# Autodesk Inventor assembly: Ensamble eléctrico
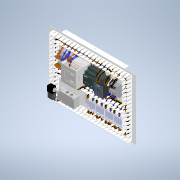
[picture p0: Inventor's stored thumbnail of the model, 180x180]
Saved by Autodesk Inventor 2021 (Build 250183000, 183)
## iProperties
Created: 2021-04-14
Part Number: Ensamble eléctrico
Document SubType Name: Assembly
Designer: Nelson
Mass: 3673.58 g
Surface Area: 11945 cm^2
Volume: 1889.25 cm^3
Density: 1.94447 g/cm^3
Author: Nelson
## Documents named in this file (23)
- C:\Users\Nelson\Github\Proyecto_PAI_2021\01 CAD\Ensamble eléctrico.iam
- C:\Users\Nelson\Github\Proyecto_PAI_2021\01 CAD\PLC-CP1E_N20DT1_D.iam
- C:\Users\Nelson\Github\Proyecto_PAI_2021\01 CAD\FuenteDC.iam
- C:\Users\Nelson\Github\Proyecto_PAI_2021\01 CAD\Rele de estado solido.ipt
- C:\Users\Nelson\Github\Proyecto_PAI_2021\01 CAD\Portafusible para fusible de 2A.ipt
- C:\Users\Nelson\Github\Proyecto_PAI_2021\01 CAD\Contactor.ipt
- C:\Users\Nelson\Github\Proyecto_PAI_2021\01 CAD\Riel 35x7.5 378mm.ipt
- C:\Users\Nelson\Github\Proyecto_PAI_2021\01 CAD\Bornera_AC.ipt
- C:\Users\Nelson\Github\Proyecto_PAI_2021\01 CAD\Bornera_DC.ipt
- C:\Users\Nelson\Github\Proyecto_PAI_2021\01 CAD\Canaleta 30x30 438mm.iam
- C:\Users\Nelson\Github\Proyecto_PAI_2021\01 CAD\Canaleta 30x30 378mm.iam
- C:\Users\Nelson\Github\Proyecto_PAI_2021\01 CAD\Canaleta 30x30 317mm.iam
- C:\Users\Nelson\Github\Proyecto_PAI_2021\01 CAD\Tapa_interior_1b.ipt
- C:\Users\Nelson\Github\Proyecto_PAI_2021\01 CAD\DIN EN ISO 7049 - ST4,8 x 13 - C - H.ipt
- C:\Users\Nelson\Github\Proyecto_PAI_2021\01 CAD\Ensamble electroválvula y bobina.iam
- C:\Users\Nelson\Github\Proyecto_PAI_2021\01 CAD\Fusible de 2A.ipt
- C:\Users\Nelson\Github\Proyecto_PAI_2021\01 CAD\Base Valvula.ipt
- C:\Users\Nelson\Github\Proyecto_PAI_2021\01 CAD\DIN EN ISO 7049 - ST4,8 x 38 - C - H.ipt
- C:\Users\Nelson\Github\Proyecto_PAI_2021\01 CAD\v70ss004001.iam
- C:\Users\Nelson\Github\Proyecto_PAI_2021\01 CAD\SV1.25-4S.ipt
- C:\Users\Nelson\Github\Proyecto_PAI_2021\01 CAD\v70ss004002.iam
- C:\Users\Nelson\Github\Proyecto_PAI_2021\01 CAD\Ensamble eléctrico\AIP\Cable and Harness\Ensamble eléctrico.Harness1.iam
- C:\Users\Nelson\Github\Proyecto_PAI_2021\01 CAD\1-34243-1.ipt
## Components (137 placed, 22 different names)
1. PLC-CP1E_N20DT1_D:1 [sub-assembly] — Mate:13, Mate:14, Mate:147, Mate:148, Mate:249, Mate:250, Mate:251, Mate:252, Mate:253, Mate:254, Mate:255, Mate:256, Mate:260, Mate:261, Mate:262, Mate:263, Mate:378, Mate:379, Mate:380, Mate:381, Mate:382, Mate:383, Mate:384, Mate:385, Mate:386, Mate:387, Mate:388, Mate:389, Mate:390, Mate:391, Mate:392, Mate:393, Mate:394, Mate:395, Mate:396, Mate:397, Mate:398, Mate:399, Mate:401, Mate:402, Mate:403, Mate:404, Mate:405, Mate:406, Mate:407, Mate:408, Mate:409, Mate:410, Mate:411
2. FuenteDC:1 [sub-assembly] — Mate:15, Mate:16, Mate:148, Mate:149, Mate:243, Mate:244, Mate:245, Mate:246, Mate:247, Mate:248, Mate:364, Mate:365, Mate:366, Mate:367, Mate:368, Mate:369
3. Portafusible para fusible de 2A:1 — Mate:17, Mate:18, Mate:149, Mate:150, Mate:204, Mate:205, Mate:360, Mate:361, Mate:362, Mate:363
4. Contactor:1 — Mate:19, Mate:20, Mate:150, Mate:151, Mate:370, Mate:371, Mate:372, Mate:373, Mate:374, Mate:375, Mate:376, Mate:377
5. Riel 35x7.5 378mm:1 — Mate:13, Mate:14, Mate:15, Mate:16, Mate:17, Mate:18, Mate:19, Mate:20, Mate:21, Mate:22, Mate:23, Mate:24, Mate:26, Mate:27, Mate:28, Mate:29, Mate:31, Mate:32, Mate:34, Mate:35, Mate:37, Mate:38, Mate:39, Mate:40, Mate:42, Mate:43, Mate:45, Mate:46, Mate:48, Mate:49, Mate:87, Mate:96, Mate:97, Flush:45, Mate:141, Mate:143, Mate:145, Mate:294, Mate:295, Mate:296, Mate:297, Mate:298, Mate:299, Mate:300, Mate:301
6. Bornera_AC:1 — Mate:21, Mate:22, Mate:25, Mate:151, Mate:338, Mate:339, Mate:343, Mate:359
7. Bornera_AC:2 — Mate:23, Mate:24, Mate:25, Mate:305, Mate:340, Mate:341, Mate:344, Mate:358
8. Bornera_DC:1 — Mate:26, Mate:27, Mate:30, Mate:89, Mate:215, Mate:222
9. Bornera_DC:2 — Mate:28, Mate:29, Mate:30, Mate:33, Mate:211, Mate:214, Mate:218, Mate:221
10. Bornera_DC:3 — Mate:31, Mate:32, Mate:33, Mate:36, Mate:210, Mate:213, Mate:217, Mate:220
11. Bornera_DC:4 — Mate:34, Mate:35, Mate:36, Mate:146, Mate:209, Mate:212, Mate:216, Mate:219
12. Bornera_DC:5 — Mate:39, Mate:40, Mate:41, Mate:44, Mate:226, Mate:231, Mate:236, Mate:241
13. Bornera_DC:6 — Mate:42, Mate:43, Mate:44, Mate:47, Mate:225, Mate:230, Mate:235, Mate:240
14. Bornera_DC:7 — Mate:45, Mate:46, Mate:47, Mate:50, Mate:224, Mate:229, Mate:234, Mate:239
15. Bornera_DC:8 — Mate:48, Mate:49, Mate:50, Mate:89, Mate:223, Mate:228, Mate:233, Mate:238
16. Bornera_DC:9 — Mate:37, Mate:38, Mate:41, Mate:147, Mate:227, Mate:232, Mate:237, Mate:242
17. Canaleta 30x30 438mm:1 [sub-assembly] — Mate:79, Mate:83, Mate:96, Flush:41, Mate:109, Flush:53, Mate:116, Mate:117, Mate:118, Mate:119, Mate:120, Mate:121
18. Canaleta 30x30 317mm:1 [sub-assembly] — Mate:79, Mate:81, Mate:87, Mate:94, Flush:41, Flush:42, Flush:54, Mate:110, Mate:111, Mate:112, Mate:113, Mate:114, Mate:115, Mate:146
19. Canaleta 30x30 438mm:2 [sub-assembly] — Mate:81, Mate:84, Flush:42, Flush:43, Mate:128, Mate:129, Mate:130, Mate:131, Mate:132, Mate:133, Mate:412, Flush:57, Mate:413, Flush:58, Mate:414, Mate:415
20. Canaleta 30x30 317mm:2 [sub-assembly] — Mate:83, Mate:84, Flush:43, Flush:44, Flush:45, Mate:122, Mate:123, Mate:124, Mate:125, Mate:126, Mate:127
21. Canaleta 30x30 378mm:1 [sub-assembly] — Mate:94, Mate:97, Flush:44, Mate:134, Mate:135, Mate:136, Mate:137, Mate:138, Mate:139
22. Tapa_interior_1b:1 — Flush:51, Flush:52, Mate:109, Flush:53, Flush:54, Mate:140, Mate:177, Mate:178, Mate:179, Mate:180, Mate:181, Mate:182, Mate:183, Mate:184, Mate:185, Mate:186, Mate:187, Mate:188, Coincidencia:206
23. DIN EN ISO 7049 - C-H ST4,8 x 13 - C - H:1 — Mate:110, Mate:111
24. DIN EN ISO 7049 - C-H ST4,8 x 13 - C - H:2 — Mate:112, Mate:113
25. DIN EN ISO 7049 - C-H ST4,8 x 13 - C - H:3 — Mate:114, Mate:115
26. DIN EN ISO 7049 - C-H ST4,8 x 13 - C - H:4 — Mate:122, Mate:123
27. DIN EN ISO 7049 - C-H ST4,8 x 13 - C - H:5 — Mate:124, Mate:125
28. DIN EN ISO 7049 - C-H ST4,8 x 13 - C - H:6 — Mate:126, Mate:127
29. DIN EN ISO 7049 - C-H ST4,8 x 13 - C - H:7 — Mate:132, Mate:133
30. DIN EN ISO 7049 - C-H ST4,8 x 13 - C - H:8 — Mate:130, Mate:131
31. DIN EN ISO 7049 - C-H ST4,8 x 13 - C - H:9 — Mate:128, Mate:129
32. DIN EN ISO 7049 - C-H ST4,8 x 13 - C - H:10 — Mate:116, Mate:117
33. DIN EN ISO 7049 - C-H ST4,8 x 13 - C - H:11 — Mate:118, Mate:119
34. DIN EN ISO 7049 - C-H ST4,8 x 13 - C - H:12 — Mate:120, Mate:121
35. DIN EN ISO 7049 - C-H ST4,8 x 13 - C - H:13 — Mate:138, Mate:139
36. DIN EN ISO 7049 - C-H ST4,8 x 13 - C - H:14 — Mate:136, Mate:137
37. DIN EN ISO 7049 - C-H ST4,8 x 13 - C - H:15 — Mate:134, Mate:135
38. DIN EN ISO 7049 - C-H ST4,8 x 13 - C - H:16 — Mate:140, Mate:141
39. DIN EN ISO 7049 - C-H ST4,8 x 13 - C - H:17 — Mate:143
40. DIN EN ISO 7049 - C-H ST4,8 x 13 - C - H:18 — Mate:145
41. Rele de estado solido:1 — Mate:177, Mate:178, Mate:179, Mate:189, Mate:190, Mate:191, Mate:192, Mate:306, Mate:307, Mate:314, Mate:315, Mate:322, Mate:323, Mate:336, Mate:337
42. Rele de estado solido:2 — Mate:180, Mate:181, Mate:182, Mate:193, Mate:194, Mate:195, Mate:308, Mate:309, Mate:316, Mate:317, Mate:324, Mate:325, Mate:334, Mate:335
43. Rele de estado solido:3 — Mate:183, Mate:184, Mate:185, Mate:196, Mate:197, Mate:198, Mate:199, Mate:310, Mate:311, Mate:318, Mate:319, Mate:326, Mate:327, Mate:332, Mate:333
44. Rele de estado solido:4 — Mate:186, Mate:187, Mate:188, Mate:200, Mate:201, Mate:202, Mate:203, Mate:312, Mate:313, Mate:320, Mate:321, Mate:328, Mate:329, Mate:330, Mate:331
45. DIN EN ISO 7049 - C-H ST4,8 x 13 - C - H:19 — Mate:189, Mate:190
46. DIN EN ISO 7049 - C-H ST4,8 x 13 - C - H:20 — Mate:191, Mate:192
47. DIN EN ISO 7049 - C-H ST4,8 x 13 - C - H:21 — Mate:193, Mate:194
48. DIN EN ISO 7049 - C-H ST4,8 x 13 - C - H:22 — Mate:195
49. DIN EN ISO 7049 - C-H ST4,8 x 13 - C - H:23 — Mate:196, Mate:197
50. DIN EN ISO 7049 - C-H ST4,8 x 13 - C - H:24 — Mate:198, Mate:199
51. DIN EN ISO 7049 - C-H ST4,8 x 13 - C - H:25 — Mate:200, Mate:201
52. DIN EN ISO 7049 - C-H ST4,8 x 13 - C - H:26 — Mate:202, Mate:203
53. Fusible de 2A:1 — Mate:204, Mate:205
54. Ensamble electroválvula y bobina:2 [sub-assembly] — Coincidencia:207, Nivelación:56, Coincidencia:208, De rotación:5, De rotación:6
55. Base Valvula:1 — Coincidencia:206, Coincidencia:207, Nivelación:56, Coincidencia:208, De rotación:1, De rotación:2, De rotación:3, De rotación:4
56. DIN EN ISO 7049 - C-H ST4,8 x 13 - C - H:27 — De rotación:1
57. DIN EN ISO 7049 - C-H ST4,8 x 13 - C - H:28 — De rotación:2
58. DIN EN ISO 7049 - C-H ST4,8 x 13 - C - H:29 — De rotación:4
59. DIN EN ISO 7049 - C-H ST4,8 x 13 - C - H:30 — De rotación:3
60. DIN EN ISO 7049 - C-H ST4,8 x 38 - C - H:1 — De rotación:6
61. DIN EN ISO 7049 - C-H ST4,8 x 38 - C - H:2 — De rotación:5
62. v70ss004001:1 [sub-assembly] — Mate:209, Mate:216
63. v70ss004001:2 [sub-assembly] — Mate:210, Mate:217
64. v70ss004001:3 [sub-assembly] — Mate:211, Mate:218
65. v70ss004001:4 [sub-assembly] — Mate:215, Mate:222
66. v70ss004001:5 [sub-assembly] — Mate:213, Mate:220
67. v70ss004001:6 [sub-assembly] — Mate:212, Mate:219
68. v70ss004001:7 [sub-assembly] — Mate:214, Mate:221
69. v70ss004001:8 [sub-assembly] — Mate:225, Mate:235
70. v70ss004001:9 [sub-assembly] — Mate:226, Mate:236
71. v70ss004001:10 [sub-assembly] — Mate:227, Mate:237
72. v70ss004001:11 [sub-assembly] — Mate:230, Mate:240
73. v70ss004001:12 [sub-assembly] — Mate:231, Mate:241
74. v70ss004001:13 [sub-assembly] — Mate:232, Mate:242
75. v70ss004001:14 [sub-assembly] — Mate:224, Mate:234
76. v70ss004001:15 [sub-assembly] — Mate:223, Mate:233
77. v70ss004001:16 [sub-assembly] — Mate:229, Mate:239
78. v70ss004001:17 [sub-assembly] — Mate:228, Mate:238
79. v70ss004001:19 [sub-assembly] — Mate:243, Mate:244, Mate:245
80. v70ss004001:20 [sub-assembly] — Mate:246, Mate:247, Mate:248
81. SV1.25-4S:3 — Mate:252, Mate:256, Mate:263
82. SV1.25-4S:10 — Mate:251, Mate:255, Mate:262
83. SV1.25-4S:11 — Mate:249, Mate:253, Mate:260
84. SV1.25-4S:12 — Mate:250, Mate:254, Mate:261
85. Bornera_AC:3 — Mate:294, Mate:298, Mate:304, Mate:305, Mate:342, Mate:345, Mate:351, Mate:357
86. Bornera_AC:4 — Mate:295, Mate:299, Mate:303, Mate:304, Mate:346, Mate:349, Mate:352, Mate:356
87. Bornera_AC:5 — Mate:296, Mate:300, Mate:302, Mate:303, Mate:347, Mate:350, Mate:353, Mate:355
88. Bornera_AC:6 — Mate:297, Mate:301, Mate:302, Mate:348, Mate:354
89. SV1.25-4S:24 — Mate:306, Mate:314
90. SV1.25-4S:25 — Mate:307, Mate:315
91. SV1.25-4S:26 — Mate:308, Mate:316
92. SV1.25-4S:27 — Mate:309, Mate:317
93. SV1.25-4S:28 — Mate:310, Mate:318
94. SV1.25-4S:29 — Mate:311, Mate:319
95. SV1.25-4S:30 — Mate:312, Mate:320
96. SV1.25-4S:31 — Mate:313, Mate:321
97. SV1.25-4S:33 — Mate:322, Mate:337
98. SV1.25-4S:34 — Mate:323, Mate:336
99. SV1.25-4S:35 — Mate:324, Mate:335
100. SV1.25-4S:36 — Mate:325, Mate:334
101. SV1.25-4S:37 — Mate:326, Mate:333
102. SV1.25-4S:38 — Mate:327, Mate:332
103. SV1.25-4S:39 — Mate:328, Mate:331
104. SV1.25-4S:40 — Mate:329, Mate:330
105. v70ss004002:1 [sub-assembly] — Mate:340, Mate:341
106. v70ss004002:2 [sub-assembly] — Mate:338, Mate:339
107. v70ss004002:3 [sub-assembly] — Mate:342, Mate:351
108. v70ss004002:4 [sub-assembly] — Mate:350, Mate:353
109. v70ss004002:5 [sub-assembly] — Mate:349, Mate:352
110. v70ss004002:6 [sub-assembly] — Mate:343, Mate:359
111. v70ss004002:7 [sub-assembly] — Mate:344, Mate:358
112. v70ss004002:8 [sub-assembly] — Mate:345, Mate:357
113. v70ss004002:9 [sub-assembly] — Mate:346, Mate:356
114. v70ss004002:10 [sub-assembly] — Mate:347, Mate:355
115. v70ss004002:11 [sub-assembly] — Mate:348, Mate:354
116. v70ss004002:12 [sub-assembly] — Mate:361, Mate:363
117. v70ss004002:13 [sub-assembly] — Mate:360, Mate:362
118. v70ss004002:14 [sub-assembly] — Mate:364, Mate:366, Mate:368
119. v70ss004002:15 [sub-assembly] — Mate:365, Mate:367, Mate:369
120. SV1.25-4S:41 — Mate:370, Mate:371
121. SV1.25-4S:42 — Mate:372, Mate:373
122. SV1.25-4S:43 — Mate:374, Mate:377
123. SV1.25-4S:44 — Mate:375, Mate:376
124. Harness1 [sub-assembly]
125. SV1.25-4S:45 — Mate:383, Mate:394, Mate:405
126. SV1.25-4S:46 — Mate:382, Mate:393, Mate:404
127. SV1.25-4S:47 — Mate:381, Mate:392, Mate:403
128. SV1.25-4S:48 — Mate:388, Mate:399, Mate:410
129. SV1.25-4S:49 — Mate:380, Mate:391, Mate:402
130. SV1.25-4S:50 — Mate:379, Mate:390, Mate:401
131. SV1.25-4S:51 — Mate:378, Mate:389, Mate:411
132. SV1.25-4S:52 — Mate:384, Mate:395, Mate:406
133. SV1.25-4S:53 — Mate:385, Mate:396, Mate:407
134. SV1.25-4S:54 — Mate:386, Mate:397, Mate:408
135. SV1.25-4S:55 — Mate:387, Mate:398, Mate:409
136. 1-34243-1:1 — Mate:413, Flush:58, Mate:415
137. 1-34243-1:2 — Mate:412, Flush:57, Mate:414
## Relationships (311: Mate 293, Flush 12, RevoluteJoint 6)
- Mate:13: PLC-CP1E_N20DT1_D:1 ↔ Riel 35x7.5 378mm:1
- Mate:14: PLC-CP1E_N20DT1_D:1 ↔ Riel 35x7.5 378mm:1
- Mate:15: FuenteDC:1 ↔ Riel 35x7.5 378mm:1
- Mate:16: FuenteDC:1 ↔ Riel 35x7.5 378mm:1
- Mate:17: Portafusible para fusible de 2A:1 ↔ Riel 35x7.5 378mm:1
- Mate:18: Portafusible para fusible de 2A:1 ↔ Riel 35x7.5 378mm:1
- Mate:19: Contactor:1 ↔ Riel 35x7.5 378mm:1
- Mate:20: Contactor:1 ↔ Riel 35x7.5 378mm:1
- Mate:21: Riel 35x7.5 378mm:1 ↔ Bornera_AC:1
- Mate:22: Riel 35x7.5 378mm:1 ↔ Bornera_AC:1
- Mate:23: Riel 35x7.5 378mm:1 ↔ Bornera_AC:2
- Mate:24: Riel 35x7.5 378mm:1 ↔ Bornera_AC:2
- Mate:25: Bornera_AC:1 ↔ Bornera_AC:2
- Mate:26: Riel 35x7.5 378mm:1 ↔ Bornera_DC:1
- Mate:27: Riel 35x7.5 378mm:1 ↔ Bornera_DC:1
- Mate:28: Riel 35x7.5 378mm:1 ↔ Bornera_DC:2
- Mate:29: Riel 35x7.5 378mm:1 ↔ Bornera_DC:2
- Mate:30: Bornera_DC:1 ↔ Bornera_DC:2
- Mate:31: Riel 35x7.5 378mm:1 ↔ Bornera_DC:3
- Mate:32: Riel 35x7.5 378mm:1 ↔ Bornera_DC:3
- Mate:33: Bornera_DC:2 ↔ Bornera_DC:3
- Mate:34: Riel 35x7.5 378mm:1 ↔ Bornera_DC:4
- Mate:35: Riel 35x7.5 378mm:1 ↔ Bornera_DC:4
- Mate:36: Bornera_DC:3 ↔ Bornera_DC:4
- Mate:37: Riel 35x7.5 378mm:1 ↔ Bornera_DC:9
- Mate:38: Riel 35x7.5 378mm:1 ↔ Bornera_DC:9
- Mate:39: Riel 35x7.5 378mm:1 ↔ Bornera_DC:5
- Mate:40: Riel 35x7.5 378mm:1 ↔ Bornera_DC:5
- Mate:41: Bornera_DC:5 ↔ Bornera_DC:9
- Mate:42: Riel 35x7.5 378mm:1 ↔ Bornera_DC:6
- Mate:43: Riel 35x7.5 378mm:1 ↔ Bornera_DC:6
- Mate:44: Bornera_DC:5 ↔ Bornera_DC:6
- Mate:45: Riel 35x7.5 378mm:1 ↔ Bornera_DC:7
- Mate:46: Riel 35x7.5 378mm:1 ↔ Bornera_DC:7
- Mate:47: Bornera_DC:6 ↔ Bornera_DC:7
- Mate:48: Riel 35x7.5 378mm:1 ↔ Bornera_DC:8
- Mate:49: Riel 35x7.5 378mm:1 ↔ Bornera_DC:8
- Mate:50: Bornera_DC:7 ↔ Bornera_DC:8
- Mate:79: Canaleta 30x30 438mm:1 ↔ Canaleta 30x30 317mm:1
- Mate:81: Canaleta 30x30 317mm:1 ↔ Canaleta 30x30 438mm:2
- Mate:83: Canaleta 30x30 438mm:1 ↔ Canaleta 30x30 317mm:2
- Mate:84: Canaleta 30x30 438mm:2 ↔ Canaleta 30x30 317mm:2
- Mate:87: Riel 35x7.5 378mm:1 ↔ Canaleta 30x30 317mm:1
- Mate:89 (7 mm): Bornera_DC:1 ↔ Bornera_DC:8
- Mate:94: Canaleta 30x30 317mm:1 ↔ Canaleta 30x30 378mm:1
- Mate:96 (47 mm): Riel 35x7.5 378mm:1 ↔ Canaleta 30x30 438mm:1
- Mate:97 (48 mm): Riel 35x7.5 378mm:1 ↔ Canaleta 30x30 378mm:1
- Flush:41: Canaleta 30x30 438mm:1 ↔ Canaleta 30x30 317mm:1
- Flush:42: Canaleta 30x30 317mm:1 ↔ Canaleta 30x30 438mm:2
- Flush:43: Canaleta 30x30 438mm:2 ↔ Canaleta 30x30 317mm:2
- Flush:44: Canaleta 30x30 317mm:2 ↔ Canaleta 30x30 378mm:1
- Flush:45: Riel 35x7.5 378mm:1 ↔ Canaleta 30x30 317mm:2
- Flush:51: Tapa_interior_1b:1
- Flush:52: Tapa_interior_1b:1
- Mate:109: Canaleta 30x30 438mm:1 ↔ Tapa_interior_1b:1
- Flush:53 (10.29 mm): Canaleta 30x30 438mm:1 ↔ Tapa_interior_1b:1
- Flush:54 (21 mm): Canaleta 30x30 317mm:1 ↔ Tapa_interior_1b:1
- Mate:110: Canaleta 30x30 317mm:1 ↔ DIN EN ISO 7049 - C-H ST4,8 x 13 - C - H:1
- Mate:111: Canaleta 30x30 317mm:1 ↔ DIN EN ISO 7049 - C-H ST4,8 x 13 - C - H:1
- Mate:112: Canaleta 30x30 317mm:1 ↔ DIN EN ISO 7049 - C-H ST4,8 x 13 - C - H:2
- Mate:113: Canaleta 30x30 317mm:1 ↔ DIN EN ISO 7049 - C-H ST4,8 x 13 - C - H:2
- Mate:114: Canaleta 30x30 317mm:1 ↔ DIN EN ISO 7049 - C-H ST4,8 x 13 - C - H:3
- Mate:115: Canaleta 30x30 317mm:1 ↔ DIN EN ISO 7049 - C-H ST4,8 x 13 - C - H:3
- Mate:116: Canaleta 30x30 438mm:1 ↔ DIN EN ISO 7049 - C-H ST4,8 x 13 - C - H:10
- Mate:117: Canaleta 30x30 438mm:1 ↔ DIN EN ISO 7049 - C-H ST4,8 x 13 - C - H:10
- Mate:118: Canaleta 30x30 438mm:1 ↔ DIN EN ISO 7049 - C-H ST4,8 x 13 - C - H:11
- Mate:119: Canaleta 30x30 438mm:1 ↔ DIN EN ISO 7049 - C-H ST4,8 x 13 - C - H:11
- Mate:120: Canaleta 30x30 438mm:1 ↔ DIN EN ISO 7049 - C-H ST4,8 x 13 - C - H:12
- Mate:121: Canaleta 30x30 438mm:1 ↔ DIN EN ISO 7049 - C-H ST4,8 x 13 - C - H:12
- Mate:122: Canaleta 30x30 317mm:2 ↔ DIN EN ISO 7049 - C-H ST4,8 x 13 - C - H:4
- Mate:123: Canaleta 30x30 317mm:2 ↔ DIN EN ISO 7049 - C-H ST4,8 x 13 - C - H:4
- Mate:124: Canaleta 30x30 317mm:2 ↔ DIN EN ISO 7049 - C-H ST4,8 x 13 - C - H:5
- Mate:125: Canaleta 30x30 317mm:2 ↔ DIN EN ISO 7049 - C-H ST4,8 x 13 - C - H:5
- Mate:126: Canaleta 30x30 317mm:2 ↔ DIN EN ISO 7049 - C-H ST4,8 x 13 - C - H:6
- Mate:127: Canaleta 30x30 317mm:2 ↔ DIN EN ISO 7049 - C-H ST4,8 x 13 - C - H:6
- Mate:128: Canaleta 30x30 438mm:2 ↔ DIN EN ISO 7049 - C-H ST4,8 x 13 - C - H:9
- Mate:129: Canaleta 30x30 438mm:2 ↔ DIN EN ISO 7049 - C-H ST4,8 x 13 - C - H:9
- Mate:130: Canaleta 30x30 438mm:2 ↔ DIN EN ISO 7049 - C-H ST4,8 x 13 - C - H:8
- Mate:131: Canaleta 30x30 438mm:2 ↔ DIN EN ISO 7049 - C-H ST4,8 x 13 - C - H:8
- Mate:132: Canaleta 30x30 438mm:2 ↔ DIN EN ISO 7049 - C-H ST4,8 x 13 - C - H:7
- Mate:133: Canaleta 30x30 438mm:2 ↔ DIN EN ISO 7049 - C-H ST4,8 x 13 - C - H:7
- Mate:134: Canaleta 30x30 378mm:1 ↔ DIN EN ISO 7049 - C-H ST4,8 x 13 - C - H:15
- Mate:135: Canaleta 30x30 378mm:1 ↔ DIN EN ISO 7049 - C-H ST4,8 x 13 - C - H:15
- Mate:136: Canaleta 30x30 378mm:1 ↔ DIN EN ISO 7049 - C-H ST4,8 x 13 - C - H:14
- Mate:137: Canaleta 30x30 378mm:1 ↔ DIN EN ISO 7049 - C-H ST4,8 x 13 - C - H:14
- Mate:138: Canaleta 30x30 378mm:1 ↔ DIN EN ISO 7049 - C-H ST4,8 x 13 - C - H:13
- Mate:139: Canaleta 30x30 378mm:1 ↔ DIN EN ISO 7049 - C-H ST4,8 x 13 - C - H:13
- Mate:140: Tapa_interior_1b:1 ↔ DIN EN ISO 7049 - C-H ST4,8 x 13 - C - H:16
- Mate:141: Riel 35x7.5 378mm:1 ↔ DIN EN ISO 7049 - C-H ST4,8 x 13 - C - H:16
- Mate:143: Riel 35x7.5 378mm:1 ↔ DIN EN ISO 7049 - C-H ST4,8 x 13 - C - H:17
- Mate:145: Riel 35x7.5 378mm:1 ↔ DIN EN ISO 7049 - C-H ST4,8 x 13 - C - H:18
- Mate:146 (28 mm): Bornera_DC:4 ↔ Canaleta 30x30 317mm:1
- Mate:147 (7 mm): PLC-CP1E_N20DT1_D:1 ↔ Bornera_DC:9
- Mate:148 (11 mm): PLC-CP1E_N20DT1_D:1 ↔ FuenteDC:1
- Mate:149 (5 mm): FuenteDC:1 ↔ Portafusible para fusible de 2A:1
- Mate:150 (5 mm): Portafusible para fusible de 2A:1 ↔ Contactor:1
- Mate:151 (5 mm): Contactor:1 ↔ Bornera_AC:1
- Mate:177: Tapa_interior_1b:1 ↔ Rele de estado solido:1
- Mate:178: Tapa_interior_1b:1 ↔ Rele de estado solido:1
- Mate:179: Tapa_interior_1b:1 ↔ Rele de estado solido:1
- Mate:180: Tapa_interior_1b:1 ↔ Rele de estado solido:2
- Mate:181: Tapa_interior_1b:1 ↔ Rele de estado solido:2
- Mate:182: Tapa_interior_1b:1 ↔ Rele de estado solido:2
- Mate:183: Tapa_interior_1b:1 ↔ Rele de estado solido:3
- Mate:184: Tapa_interior_1b:1 ↔ Rele de estado solido:3
- Mate:185: Tapa_interior_1b:1 ↔ Rele de estado solido:3
- Mate:186: Tapa_interior_1b:1 ↔ Rele de estado solido:4
- Mate:187: Tapa_interior_1b:1 ↔ Rele de estado solido:4
- Mate:188: Tapa_interior_1b:1 ↔ Rele de estado solido:4
- Mate:189: Rele de estado solido:1 ↔ DIN EN ISO 7049 - C-H ST4,8 x 13 - C - H:19
- Mate:190: Rele de estado solido:1 ↔ DIN EN ISO 7049 - C-H ST4,8 x 13 - C - H:19
- Mate:191: Rele de estado solido:1 ↔ DIN EN ISO 7049 - C-H ST4,8 x 13 - C - H:20
- Mate:192: Rele de estado solido:1 ↔ DIN EN ISO 7049 - C-H ST4,8 x 13 - C - H:20
- Mate:193: Rele de estado solido:2 ↔ DIN EN ISO 7049 - C-H ST4,8 x 13 - C - H:21
- Mate:194: Rele de estado solido:2 ↔ DIN EN ISO 7049 - C-H ST4,8 x 13 - C - H:21
- Mate:195: Rele de estado solido:2 ↔ DIN EN ISO 7049 - C-H ST4,8 x 13 - C - H:22
- Mate:196: Rele de estado solido:3 ↔ DIN EN ISO 7049 - C-H ST4,8 x 13 - C - H:23
- Mate:197: Rele de estado solido:3 ↔ DIN EN ISO 7049 - C-H ST4,8 x 13 - C - H:23
- Mate:198: Rele de estado solido:3 ↔ DIN EN ISO 7049 - C-H ST4,8 x 13 - C - H:24
- Mate:199: Rele de estado solido:3 ↔ DIN EN ISO 7049 - C-H ST4,8 x 13 - C - H:24
- Mate:200: Rele de estado solido:4 ↔ DIN EN ISO 7049 - C-H ST4,8 x 13 - C - H:25
- Mate:201: Rele de estado solido:4 ↔ DIN EN ISO 7049 - C-H ST4,8 x 13 - C - H:25
- Mate:202: Rele de estado solido:4 ↔ DIN EN ISO 7049 - C-H ST4,8 x 13 - C - H:26
- Mate:203: Rele de estado solido:4 ↔ DIN EN ISO 7049 - C-H ST4,8 x 13 - C - H:26
- Mate:204: Portafusible para fusible de 2A:1 ↔ Fusible de 2A:1
- Mate:205: Portafusible para fusible de 2A:1 ↔ Fusible de 2A:1
- Coincidencia:206 [Mate]: Tapa_interior_1b:1 ↔ Base Valvula:1
- Coincidencia:207 [Mate]: Ensamble electroválvula y bobina:2 ↔ Base Valvula:1
- Nivelación:56 [Flush]: Ensamble electroválvula y bobina:2 ↔ Base Valvula:1
- Coincidencia:208 [Mate]: Ensamble electroválvula y bobina:2 ↔ Base Valvula:1
- De rotación:1 [RevoluteJoint]: Base Valvula:1 ↔ DIN EN ISO 7049 - C-H ST4,8 x 13 - C - H:27
- De rotación:2 [RevoluteJoint]: Base Valvula:1 ↔ DIN EN ISO 7049 - C-H ST4,8 x 13 - C - H:28
- De rotación:3 [RevoluteJoint]: Base Valvula:1 ↔ DIN EN ISO 7049 - C-H ST4,8 x 13 - C - H:30
- De rotación:4 [RevoluteJoint]: Base Valvula:1 ↔ DIN EN ISO 7049 - C-H ST4,8 x 13 - C - H:29
- De rotación:5 [RevoluteJoint]: Ensamble electroválvula y bobina:2 ↔ DIN EN ISO 7049 - C-H ST4,8 x 38 - C - H:2
- De rotación:6 [RevoluteJoint]: Ensamble electroválvula y bobina:2 ↔ DIN EN ISO 7049 - C-H ST4,8 x 38 - C - H:1
- Mate:209: Bornera_DC:4 ↔ v70ss004001:1
- Mate:210: Bornera_DC:3 ↔ v70ss004001:2
- Mate:211: Bornera_DC:2 ↔ v70ss004001:3
- Mate:212: Bornera_DC:4 ↔ v70ss004001:6
- Mate:213: Bornera_DC:3 ↔ v70ss004001:5
- Mate:214: Bornera_DC:2 ↔ v70ss004001:7
- Mate:215: Bornera_DC:1 ↔ v70ss004001:4
- Mate:216: Bornera_DC:4 ↔ v70ss004001:1
- Mate:217: Bornera_DC:3 ↔ v70ss004001:2
- Mate:218: Bornera_DC:2 ↔ v70ss004001:3
- Mate:219: Bornera_DC:4 ↔ v70ss004001:6
- Mate:220: Bornera_DC:3 ↔ v70ss004001:5
- Mate:221: Bornera_DC:2 ↔ v70ss004001:7
- Mate:222: Bornera_DC:1 ↔ v70ss004001:4
- Mate:223: Bornera_DC:8 ↔ v70ss004001:15
- Mate:224: Bornera_DC:7 ↔ v70ss004001:14
- Mate:225: Bornera_DC:6 ↔ v70ss004001:8
- Mate:226: Bornera_DC:5 ↔ v70ss004001:9
- Mate:227: Bornera_DC:9 ↔ v70ss004001:10
- Mate:228: Bornera_DC:8 ↔ v70ss004001:17
- Mate:229: Bornera_DC:7 ↔ v70ss004001:16
- Mate:230: Bornera_DC:6 ↔ v70ss004001:11
- Mate:231: Bornera_DC:5 ↔ v70ss004001:12
- Mate:232: Bornera_DC:9 ↔ v70ss004001:13
- Mate:233: Bornera_DC:8 ↔ v70ss004001:15
- Mate:234: Bornera_DC:7 ↔ v70ss004001:14
- Mate:235: Bornera_DC:6 ↔ v70ss004001:8
- Mate:236: Bornera_DC:5 ↔ v70ss004001:9
- Mate:237: Bornera_DC:9 ↔ v70ss004001:10
- Mate:238: Bornera_DC:8 ↔ v70ss004001:17
- Mate:239: Bornera_DC:7 ↔ v70ss004001:16
- Mate:240: Bornera_DC:6 ↔ v70ss004001:11
- Mate:241: Bornera_DC:5 ↔ v70ss004001:12
- Mate:242: Bornera_DC:9 ↔ v70ss004001:13
- Mate:243 (2 mm): FuenteDC:1 ↔ v70ss004001:19
- Mate:244 (2.25 mm): FuenteDC:1 ↔ v70ss004001:19
- Mate:245: FuenteDC:1 ↔ v70ss004001:19
- Mate:246 (2 mm): FuenteDC:1 ↔ v70ss004001:20
- Mate:247 (2.25 mm): FuenteDC:1 ↔ v70ss004001:20
- Mate:248: FuenteDC:1 ↔ v70ss004001:20
- Mate:249: PLC-CP1E_N20DT1_D:1 ↔ SV1.25-4S:11
- Mate:250: PLC-CP1E_N20DT1_D:1 ↔ SV1.25-4S:12
- Mate:251: PLC-CP1E_N20DT1_D:1 ↔ SV1.25-4S:10
- Mate:252: PLC-CP1E_N20DT1_D:1 ↔ SV1.25-4S:3
- Mate:253: PLC-CP1E_N20DT1_D:1 ↔ SV1.25-4S:11
- Mate:254: PLC-CP1E_N20DT1_D:1 ↔ SV1.25-4S:12
- Mate:255: PLC-CP1E_N20DT1_D:1 ↔ SV1.25-4S:10
- Mate:256: PLC-CP1E_N20DT1_D:1 ↔ SV1.25-4S:3
- Mate:260: PLC-CP1E_N20DT1_D:1 ↔ SV1.25-4S:11
- Mate:261: PLC-CP1E_N20DT1_D:1 ↔ SV1.25-4S:12
- Mate:262: PLC-CP1E_N20DT1_D:1 ↔ SV1.25-4S:10
- Mate:263: PLC-CP1E_N20DT1_D:1 ↔ SV1.25-4S:3
- Mate:294: Riel 35x7.5 378mm:1 ↔ Bornera_AC:3
- Mate:295: Riel 35x7.5 378mm:1 ↔ Bornera_AC:4
- Mate:296: Riel 35x7.5 378mm:1 ↔ Bornera_AC:5
- Mate:297: Riel 35x7.5 378mm:1 ↔ Bornera_AC:6
- Mate:298: Riel 35x7.5 378mm:1 ↔ Bornera_AC:3
- Mate:299: Riel 35x7.5 378mm:1 ↔ Bornera_AC:4
- Mate:300: Riel 35x7.5 378mm:1 ↔ Bornera_AC:5
- Mate:301: Riel 35x7.5 378mm:1 ↔ Bornera_AC:6
- Mate:302: Bornera_AC:5 ↔ Bornera_AC:6
- Mate:303: Bornera_AC:4 ↔ Bornera_AC:5
- Mate:304: Bornera_AC:3 ↔ Bornera_AC:4
- Mate:305 (7 mm): Bornera_AC:2 ↔ Bornera_AC:3
- Mate:306: Rele de estado solido:1 ↔ SV1.25-4S:24
- Mate:307: Rele de estado solido:1 ↔ SV1.25-4S:25
- Mate:308: Rele de estado solido:2 ↔ SV1.25-4S:26
- Mate:309: Rele de estado solido:2 ↔ SV1.25-4S:27
- Mate:310: Rele de estado solido:3 ↔ SV1.25-4S:28
- Mate:311: Rele de estado solido:3 ↔ SV1.25-4S:29
- Mate:312: Rele de estado solido:4 ↔ SV1.25-4S:30
- Mate:313: Rele de estado solido:4 ↔ SV1.25-4S:31
- Mate:314: Rele de estado solido:1 ↔ SV1.25-4S:24
- Mate:315: Rele de estado solido:1 ↔ SV1.25-4S:25
- Mate:316: Rele de estado solido:2 ↔ SV1.25-4S:26
- Mate:317: Rele de estado solido:2 ↔ SV1.25-4S:27
- Mate:318: Rele de estado solido:3 ↔ SV1.25-4S:28
- Mate:319: Rele de estado solido:3 ↔ SV1.25-4S:29
- Mate:320: Rele de estado solido:4 ↔ SV1.25-4S:30
- Mate:321: Rele de estado solido:4 ↔ SV1.25-4S:31
- Mate:322: Rele de estado solido:1 ↔ SV1.25-4S:33
- Mate:323: Rele de estado solido:1 ↔ SV1.25-4S:34
- Mate:324: Rele de estado solido:2 ↔ SV1.25-4S:35
- Mate:325: Rele de estado solido:2 ↔ SV1.25-4S:36
- Mate:326: Rele de estado solido:3 ↔ SV1.25-4S:37
- Mate:327: Rele de estado solido:3 ↔ SV1.25-4S:38
- Mate:328: Rele de estado solido:4 ↔ SV1.25-4S:39
- Mate:329: Rele de estado solido:4 ↔ SV1.25-4S:40
- Mate:330: Rele de estado solido:4 ↔ SV1.25-4S:40
- Mate:331: Rele de estado solido:4 ↔ SV1.25-4S:39
- Mate:332: Rele de estado solido:3 ↔ SV1.25-4S:38
- Mate:333: Rele de estado solido:3 ↔ SV1.25-4S:37
- Mate:334: Rele de estado solido:2 ↔ SV1.25-4S:36
- Mate:335: Rele de estado solido:2 ↔ SV1.25-4S:35
- Mate:336: Rele de estado solido:1 ↔ SV1.25-4S:34
- Mate:337: Rele de estado solido:1 ↔ SV1.25-4S:33
- Mate:338: Bornera_AC:1 ↔ v70ss004002:2
- Mate:339: Bornera_AC:1 ↔ v70ss004002:2
- Mate:340: Bornera_AC:2 ↔ v70ss004002:1
- Mate:341: Bornera_AC:2 ↔ v70ss004002:1
- Mate:342: Bornera_AC:3 ↔ v70ss004002:3
- Mate:343: Bornera_AC:1 ↔ v70ss004002:6
- Mate:344: Bornera_AC:2 ↔ v70ss004002:7
- Mate:345: Bornera_AC:3 ↔ v70ss004002:8
- Mate:346: Bornera_AC:4 ↔ v70ss004002:9
- Mate:347: Bornera_AC:5 ↔ v70ss004002:10
- Mate:348: Bornera_AC:6 ↔ v70ss004002:11
- Mate:349: Bornera_AC:4 ↔ v70ss004002:5
- Mate:350: Bornera_AC:5 ↔ v70ss004002:4
- Mate:351: Bornera_AC:3 ↔ v70ss004002:3
- Mate:352: Bornera_AC:4 ↔ v70ss004002:5
- Mate:353: Bornera_AC:5 ↔ v70ss004002:4
- Mate:354: Bornera_AC:6 ↔ v70ss004002:11
- Mate:355: Bornera_AC:5 ↔ v70ss004002:10
- Mate:356: Bornera_AC:4 ↔ v70ss004002:9
- Mate:357: Bornera_AC:3 ↔ v70ss004002:8
- Mate:358: Bornera_AC:2 ↔ v70ss004002:7
- Mate:359: Bornera_AC:1 ↔ v70ss004002:6
- Mate:360: Portafusible para fusible de 2A:1 ↔ v70ss004002:13
- Mate:361: Portafusible para fusible de 2A:1 ↔ v70ss004002:12
- Mate:362: Portafusible para fusible de 2A:1 ↔ v70ss004002:13
- Mate:363: Portafusible para fusible de 2A:1 ↔ v70ss004002:12
- Mate:364 (2.3 mm): FuenteDC:1 ↔ v70ss004002:14
- Mate:365 (1.3 mm): FuenteDC:1 ↔ v70ss004002:15
- Mate:366 (2.25 mm): FuenteDC:1 ↔ v70ss004002:14
- Mate:367 (2.25 mm): FuenteDC:1 ↔ v70ss004002:15
- Mate:368: FuenteDC:1 ↔ v70ss004002:14
- Mate:369: FuenteDC:1 ↔ v70ss004002:15
- Mate:370: Contactor:1 ↔ SV1.25-4S:41
- Mate:371: Contactor:1 ↔ SV1.25-4S:41
- Mate:372: Contactor:1 ↔ SV1.25-4S:42
- Mate:373: Contactor:1 ↔ SV1.25-4S:42
- Mate:374: Contactor:1 ↔ SV1.25-4S:43
- Mate:375: Contactor:1 ↔ SV1.25-4S:44
- Mate:376: Contactor:1 ↔ SV1.25-4S:44
- Mate:377: Contactor:1 ↔ SV1.25-4S:43
- Mate:378: PLC-CP1E_N20DT1_D:1 ↔ SV1.25-4S:51
- Mate:379: PLC-CP1E_N20DT1_D:1 ↔ SV1.25-4S:50
- Mate:380: PLC-CP1E_N20DT1_D:1 ↔ SV1.25-4S:49
- Mate:381: PLC-CP1E_N20DT1_D:1 ↔ SV1.25-4S:47
- Mate:382: PLC-CP1E_N20DT1_D:1 ↔ SV1.25-4S:46
- Mate:383: PLC-CP1E_N20DT1_D:1 ↔ SV1.25-4S:45
- Mate:384: PLC-CP1E_N20DT1_D:1 ↔ SV1.25-4S:52
- Mate:385: PLC-CP1E_N20DT1_D:1 ↔ SV1.25-4S:53
- Mate:386: PLC-CP1E_N20DT1_D:1 ↔ SV1.25-4S:54
- Mate:387: PLC-CP1E_N20DT1_D:1 ↔ SV1.25-4S:55
- Mate:388: PLC-CP1E_N20DT1_D:1 ↔ SV1.25-4S:48
- Mate:389: PLC-CP1E_N20DT1_D:1 ↔ SV1.25-4S:51
- Mate:390: PLC-CP1E_N20DT1_D:1 ↔ SV1.25-4S:50
- Mate:391: PLC-CP1E_N20DT1_D:1 ↔ SV1.25-4S:49
- Mate:392: PLC-CP1E_N20DT1_D:1 ↔ SV1.25-4S:47
- Mate:393: PLC-CP1E_N20DT1_D:1 ↔ SV1.25-4S:46
- Mate:394: PLC-CP1E_N20DT1_D:1 ↔ SV1.25-4S:45
- Mate:395: PLC-CP1E_N20DT1_D:1 ↔ SV1.25-4S:52
- Mate:396: PLC-CP1E_N20DT1_D:1 ↔ SV1.25-4S:53
- Mate:397: PLC-CP1E_N20DT1_D:1 ↔ SV1.25-4S:54
- Mate:398: PLC-CP1E_N20DT1_D:1 ↔ SV1.25-4S:55
- Mate:399: PLC-CP1E_N20DT1_D:1 ↔ SV1.25-4S:48
- Mate:401: PLC-CP1E_N20DT1_D:1 ↔ SV1.25-4S:50
- Mate:402: PLC-CP1E_N20DT1_D:1 ↔ SV1.25-4S:49
- Mate:403: PLC-CP1E_N20DT1_D:1 ↔ SV1.25-4S:47
- Mate:404: PLC-CP1E_N20DT1_D:1 ↔ SV1.25-4S:46
- Mate:405: PLC-CP1E_N20DT1_D:1 ↔ SV1.25-4S:45
- Mate:406: PLC-CP1E_N20DT1_D:1 ↔ SV1.25-4S:52
- Mate:407: PLC-CP1E_N20DT1_D:1 ↔ SV1.25-4S:53
- Mate:408: PLC-CP1E_N20DT1_D:1 ↔ SV1.25-4S:54
- Mate:409: PLC-CP1E_N20DT1_D:1 ↔ SV1.25-4S:55
- Mate:410: PLC-CP1E_N20DT1_D:1 ↔ SV1.25-4S:48
- Mate:411: PLC-CP1E_N20DT1_D:1 ↔ SV1.25-4S:51
- Mate:412 (2.5 mm): Canaleta 30x30 438mm:2 ↔ 1-34243-1:2
- Flush:57: Canaleta 30x30 438mm:2 ↔ 1-34243-1:2
- Mate:413 (2.5 mm): Canaleta 30x30 438mm:2 ↔ 1-34243-1:1
- Flush:58: Canaleta 30x30 438mm:2 ↔ 1-34243-1:1
- Mate:414 (10 mm): Canaleta 30x30 438mm:2 ↔ 1-34243-1:2
- Mate:415 (5 mm): Canaleta 30x30 438mm:2 ↔ 1-34243-1:1
